# Autodesk Inventor assembly: 中間ユニット
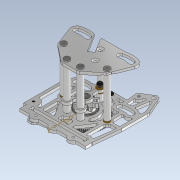
[picture p0: Inventor's stored thumbnail of the model, 180x180]
Saved by Autodesk Inventor 2020.2 (Build 242310000, 310)
## iProperties
Created: 2020-03-12
Part Number: 中間ユニット
Document SubType Name: Assembly
Designer: aoyam
Mass: 89.468 g
Surface Area: 374.989 cm^2
Volume: 27.4588 cm^3
Density: 3.25827 g/cm^3
Author: aoyam
## Documents named in this file (29)
- C:\Users\aoyam\Desktop\SRDC_local\Inventor\二年機\Geminiβ\脚\中間ユニット\中間ユニット.iam
- C:\Users\aoyam\Desktop\SRDC_local\Inventor\二年機\Geminiβ\汎用部品\ワッシャD7d3m0.5.ipt
- C:\Users\aoyam\Desktop\SRDC_local\Inventor\二年機\Geminiβ\脚\中間ユニット\中間ギア抑え.ipt
- C:\Users\aoyam\Desktop\SRDC_local\Inventor\二年機\Geminiβ\汎用部品\ベアリングd4D8B3F.ipt
- C:\Users\aoyam\Desktop\SRDC_local\Inventor\二年機\Geminiβ\汎用部品\ワッシャD7d4m0.5.ipt
- C:\Users\aoyam\Desktop\SRDC_local\Inventor\二年機\Geminiβ\汎用部品\ｍ2歯数9ギアd3.99.ipt
- C:\Users\aoyam\Desktop\SRDC_local\Inventor\二年機\Geminiβ\汎用部品\ｍ0.5歯数80ギアd15.ipt
- C:\Users\aoyam\Desktop\SRDC_local\Inventor\二年機\Geminiβ\脚\中間ユニット\脚中間フレームカム.ipt
- C:\Users\aoyam\Desktop\SRDC_local\Inventor\二年機\Geminiβ\汎用部品\ベアリングd15D21B4.ipt
- C:\Users\aoyam\Desktop\SRDC_local\Inventor\二年機\Geminiβ\脚\中間ユニット\脚中間フレームカム2.ipt
- C:\Users\aoyam\Desktop\SRDC_local\Inventor\二年機\Geminiβ\脚\中間ユニット\脚中間フレームカム3.ipt
- C:\Users\aoyam\Desktop\SRDC_local\Inventor\二年機\Geminiβ\脚\中間ユニット\中間フレーム内側.ipt
- C:\Users\aoyam\Desktop\SRDC_local\Inventor\二年機\Geminiβ\汎用部品\スペーサーM3L45アルミ.ipt
- C:\Users\aoyam\Desktop\SRDC_local\Inventor\二年機\Geminiβ\汎用部品\ネジ超極低頭M3L8.ipt
- C:\Users\aoyam\Desktop\SRDC_local\Inventor\二年機\Geminiβ\汎用部品\ネジボタンM3L6.ipt
- C:\Users\aoyam\Desktop\SRDC_local\Inventor\二年機\Geminiβ\脚\中間ユニット\モーターマウント.ipt
- C:\Users\aoyam\Desktop\SRDC_local\Inventor\二年機\Geminiβ\汎用部品\ネジボタンM3L4.ipt
- C:\Users\aoyam\Desktop\SRDC_local\Inventor\二年機\Geminiβ\汎用部品\ネジボタンM3L8.ipt
- C:\Users\aoyam\Desktop\SRDC_local\Inventor\二年機\Geminiβ\汎用部品\スペーサーM3L15アルミ.ipt
- C:\Users\aoyam\Desktop\SRDC_local\Inventor\二年機\Geminiβ\汎用部品\スペーサーM3L20アルミ.ipt
- C:\Users\aoyam\Desktop\SRDC_local\Inventor\二年機\Geminiβ\汎用部品\ネジボタンM3L10.ipt
- C:\Users\aoyam\Desktop\SRDC_local\Inventor\二年機\Geminiβ\汎用部品\スペーサー中空M3L8アルミ.ipt
- C:\Users\aoyam\Desktop\SRDC_local\Inventor\二年機\Geminiβ\汎用部品\ネジボタンM3L14.ipt
- C:\Users\aoyam\Desktop\SRDC_local\Inventor\二年機\Geminiβ\汎用部品\平行ピンD4L18.ipt
- C:\Users\aoyam\Desktop\SRDC_local\Inventor\二年機\Geminiβ\汎用部品\スペーサー中空M3L15アルミ.ipt
- C:\Users\aoyam\Desktop\SRDC_local\Inventor\二年機\Geminiβ\脚\中間ユニット\MIRright脚中間フレーム外側.ipt
- C:\Users\aoyam\Desktop\SRDC_local\Inventor\二年機\Geminiβ\汎用部品\ネジボタンM3L18.ipt
- C:\Users\aoyam\Desktop\SRDC_local\Inventor\二年機\Geminiβ\汎用部品\ワッシャD6d3m0.5.ipt
- C:\Users\aoyam\Desktop\SRDC_local\Inventor\二年機\Geminiβ\汎用部品\ネジ超低頭M3L8.ipt
## Components (50 placed, 28 different names)
1. 中間ギア抑え:1 — 挿入:5, メイト:15, 挿入:84, 挿入:85
2. ベアリングd4D8B3F:1 — 挿入:5, 挿入:6
3. ワッシャD7d4m0.5:1 — 挿入:6, 挿入:7
4. ｍ2歯数9ギアd3.99:1 — 挿入:7, メイト:3, メイト:26, メイト:27
5. ｍ0.5歯数80ギアd15:1 — 挿入:11, 挿入:47, 挿入:50, 挿入:153, 挿入:154
6. 脚中間フレームカム:1 — 挿入:10, メイト:10, 挿入:77, メイト:27
7. ベアリングd15D21B4:1 — メイト:3, 挿入:28, 挿入:79
8. 脚中間フレームカム3:1 — 挿入:10, 挿入:11, メイト:10, 挿入:153, 挿入:182, 挿入:183, 挿入:184
9. 中間フレーム内側:1 — 挿入:28, メイト:15, フラッシュ:3, メイト:22, 挿入:64, 挿入:65, 挿入:75, 挿入:89, 挿入:139, 挿入:148, 挿入:149, 挿入:164, 挿入:170, 挿入:175, 挿入:181, 挿入:185, 挿入:186, 挿入:201, 挿入:204
10. モーターマウント:1 — 挿入:134, 挿入:140, 挿入:187, 挿入:188, 挿入:207, 挿入:208
11. ネジボタンM3L4:1 — 挿入:47
12. ネジボタンM3L4:2 — 挿入:154
13. ネジボタンM3L4:4 — 挿入:50
14. ネジボタンM3L8:3 — 挿入:134
15. スペーサーM3L45アルミ:3 — メイト:22
16. ネジ超極低頭M3L8:4 — 挿入:64
17. ネジ超極低頭M3L8:5 — 挿入:65
18. ネジボタンM3L6:3 — 挿入:75
19. 脚中間フレームカム2:1 — 挿入:77, メイト:26, 挿入:79
20. スペーサーM3L45アルミ:4 — 挿入:149, 挿入:194
21. スペーサーM3L45アルミ:5 — 挿入:148, 挿入:195
22. ワッシャD7d3m0.5:2 — 挿入:84
23. ワッシャD7d3m0.5:3 — 挿入:85, 挿入:200
24. ネジボタンM3L8:4 — 挿入:89
25. スペーサーM3L45アルミ:6
26. ネジボタンM3L8:5 — 挿入:175
27. スペーサーM3L15アルミ:1 — 挿入:139, 挿入:140
28. スペーサーM3L20アルミ:1 — 挿入:164, 挿入:171
29. ネジボタンM3L6:5 — 挿入:170
30. ネジボタンM3L10:1 — 挿入:171
31. スペーサー中空M3L8アルミ:1 — 挿入:181
32. ネジボタンM3L14:1 — 挿入:182
33. ネジボタンM3L14:2 — 挿入:183
34. 平行ピンD4L18:1 — 挿入:184
35. スペーサー中空M3L15アルミ:1 — 挿入:185, 挿入:187
36. スペーサー中空M3L15アルミ:2 — 挿入:186, 挿入:188
37. MIRright脚中間フレーム外側:1 — 挿入:194, 挿入:195, 挿入:209, 挿入:210, 挿入:211, 挿入:212
38. ネジボタンM3L18:1 — 挿入:200
39. ワッシャD6d3m0.5:1 — 挿入:201, 挿入:202
40. ワッシャD6d3m0.5:2 — 挿入:202, 挿入:203
41. ワッシャD6d3m0.5:3 — 挿入:203
42. ワッシャD6d3m0.5:4 — 挿入:204, 挿入:205
43. ワッシャD6d3m0.5:5 — 挿入:205, 挿入:206
44. ワッシャD6d3m0.5:6 — 挿入:206
45. ネジボタンM3L18:2 — 挿入:207
46. ネジボタンM3L18:3 — 挿入:208
47. ネジ超低頭M3L8:1 — 挿入:212
48. ネジ超低頭M3L8:2 — 挿入:211
49. ネジ超低頭M3L8:3 — 挿入:210
50. ネジ超低頭M3L8:4 — 挿入:209
## Relationships (57: Insert 50, Mate 6, Flush 1)
- 挿入:5 [Insert]: 中間ギア抑え:1 ↔ ベアリングd4D8B3F:1
- 挿入:6 [Insert]: ベアリングd4D8B3F:1 ↔ ワッシャD7d4m0.5:1
- 挿入:7 [Insert]: ワッシャD7d4m0.5:1 ↔ ｍ2歯数9ギアd3.99:1
- メイト:3 [Mate]: ｍ2歯数9ギアd3.99:1 ↔ ベアリングd15D21B4:1
- 挿入:10 [Insert]: 脚中間フレームカム:1 ↔ 脚中間フレームカム3:1
- 挿入:11 [Insert]: ｍ0.5歯数80ギアd15:1 ↔ 脚中間フレームカム3:1
- メイト:10 [Mate]: 脚中間フレームカム:1 ↔ 脚中間フレームカム3:1
- 挿入:28 [Insert]: ベアリングd15D21B4:1 ↔ 中間フレーム内側:1
- メイト:15 [Mate]: 中間ギア抑え:1 ↔ 中間フレーム内側:1
- 挿入:47 [Insert]: ｍ0.5歯数80ギアd15:1 ↔ ネジボタンM3L4:1
- 挿入:50 [Insert]: ｍ0.5歯数80ギアd15:1 ↔ ネジボタンM3L4:4
- フラッシュ:3 [Flush] (-38 mm): 中間フレーム内側:1
- メイト:22 [Mate]: 中間フレーム内側:1 ↔ スペーサーM3L45アルミ:3
- 挿入:64 [Insert]: 中間フレーム内側:1 ↔ ネジ超極低頭M3L8:4
- 挿入:65 [Insert]: 中間フレーム内側:1 ↔ ネジ超極低頭M3L8:5
- 挿入:75 [Insert]: 中間フレーム内側:1 ↔ ネジボタンM3L6:3
- 挿入:77 [Insert]: 脚中間フレームカム:1 ↔ 脚中間フレームカム2:1
- メイト:26 [Mate]: ｍ2歯数9ギアd3.99:1 ↔ 脚中間フレームカム2:1
- 挿入:79 [Insert]: ベアリングd15D21B4:1 ↔ 脚中間フレームカム2:1
- 挿入:84 [Insert]: 中間ギア抑え:1 ↔ ワッシャD7d3m0.5:2
- 挿入:85 [Insert]: 中間ギア抑え:1 ↔ ワッシャD7d3m0.5:3
- 挿入:89 [Insert]: 中間フレーム内側:1 ↔ ネジボタンM3L8:4
- 挿入:134 [Insert]: モーターマウント:1 ↔ ネジボタンM3L8:3
- 挿入:139 [Insert]: 中間フレーム内側:1 ↔ スペーサーM3L15アルミ:1
- 挿入:140 [Insert]: モーターマウント:1 ↔ スペーサーM3L15アルミ:1
- 挿入:148 [Insert]: 中間フレーム内側:1 ↔ スペーサーM3L45アルミ:5
- 挿入:149 [Insert]: 中間フレーム内側:1 ↔ スペーサーM3L45アルミ:4
- 挿入:153 [Insert]: ｍ0.5歯数80ギアd15:1 ↔ 脚中間フレームカム3:1
- 挿入:154 [Insert]: ｍ0.5歯数80ギアd15:1 ↔ ネジボタンM3L4:2
- 挿入:164 [Insert]: 中間フレーム内側:1 ↔ スペーサーM3L20アルミ:1
- 挿入:170 [Insert]: 中間フレーム内側:1 ↔ ネジボタンM3L6:5
- 挿入:171 [Insert] (5 mm): スペーサーM3L20アルミ:1 ↔ ネジボタンM3L10:1
- 挿入:175 [Insert]: 中間フレーム内側:1 ↔ ネジボタンM3L8:5
- 挿入:181 [Insert]: 中間フレーム内側:1 ↔ スペーサー中空M3L8アルミ:1
- メイト:27 [Mate]: ｍ2歯数9ギアd3.99:1 ↔ 脚中間フレームカム:1
- 挿入:182 [Insert]: 脚中間フレームカム3:1 ↔ ネジボタンM3L14:1
- 挿入:183 [Insert]: 脚中間フレームカム3:1 ↔ ネジボタンM3L14:2
- 挿入:184 [Insert]: 脚中間フレームカム3:1 ↔ 平行ピンD4L18:1
- 挿入:185 [Insert]: 中間フレーム内側:1 ↔ スペーサー中空M3L15アルミ:1
- 挿入:186 [Insert]: 中間フレーム内側:1 ↔ スペーサー中空M3L15アルミ:2
- 挿入:187 [Insert]: モーターマウント:1 ↔ スペーサー中空M3L15アルミ:1
- 挿入:188 [Insert]: モーターマウント:1 ↔ スペーサー中空M3L15アルミ:2
- 挿入:194 [Insert]: スペーサーM3L45アルミ:4 ↔ MIRright脚中間フレーム外側:1
- 挿入:195 [Insert]: スペーサーM3L45アルミ:5 ↔ MIRright脚中間フレーム外側:1
- 挿入:200 [Insert] (3 mm): ワッシャD7d3m0.5:3 ↔ ネジボタンM3L18:1
- 挿入:201 [Insert]: 中間フレーム内側:1 ↔ ワッシャD6d3m0.5:1
- 挿入:202 [Insert]: ワッシャD6d3m0.5:1 ↔ ワッシャD6d3m0.5:2
- 挿入:203 [Insert]: ワッシャD6d3m0.5:2 ↔ ワッシャD6d3m0.5:3
- 挿入:204 [Insert]: 中間フレーム内側:1 ↔ ワッシャD6d3m0.5:4
- 挿入:205 [Insert]: ワッシャD6d3m0.5:4 ↔ ワッシャD6d3m0.5:5
- 挿入:206 [Insert]: ワッシャD6d3m0.5:5 ↔ ワッシャD6d3m0.5:6
- 挿入:207 [Insert]: モーターマウント:1 ↔ ネジボタンM3L18:2
- 挿入:208 [Insert]: モーターマウント:1 ↔ ネジボタンM3L18:3
- 挿入:209 [Insert]: MIRright脚中間フレーム外側:1 ↔ ネジ超低頭M3L8:4
- 挿入:210 [Insert]: MIRright脚中間フレーム外側:1 ↔ ネジ超低頭M3L8:3
- 挿入:211 [Insert]: MIRright脚中間フレーム外側:1 ↔ ネジ超低頭M3L8:2
- 挿入:212 [Insert]: MIRright脚中間フレーム外側:1 ↔ ネジ超低頭M3L8:1
